# Autodesk Inventor assembly: right drive
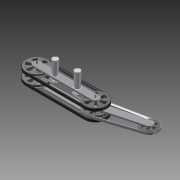
[picture p0: Inventor's stored thumbnail of the model, 180x180]
Saved by Autodesk Inventor 2011 (Build 150239000, 239)
## iProperties
Created: 2010-04-20
Part Number: right drive
Document SubType Name: Assembly
Designer: lucio
Author: lucio
## Documents named in this file (9)
- C:\Users\lucio\Documents\Inventor\caterpillar\right drive.iam
- C:\Users\lucio\Documents\Inventor\caterpillar\base side.ipt
- C:\Users\lucio\Documents\Inventor\caterpillar\mr85vel 2 etapas.ipt
- C:\Users\lucio\Documents\Inventor\caterpillar\mr85vel 3 etapas.ipt
- C:\Users\lucio\Documents\Inventor\caterpillar\back wheel.iam
- C:\Users\lucio\Documents\Inventor\caterpillar\sprocket.ipt
- C:\Users\lucio\Documents\Inventor\caterpillar\chain.ipt
- C:\Users\lucio\Documents\Inventor\caterpillar\big belt.ipt
- C:\Users\lucio\Documents\Inventor\caterpillar\outer drive side.ipt
## Components (11 placed, 8 different names)
1. base side:1 — Insert:1, Insert:2, Insert:4
2. mr85vel 2 etapas:1 — Insert:1, Mate:2, Flush:2
3. mr85vel 3 etapas:1 — Insert:2, Flush:1, Mate:1
4. back wheel:1 [sub-assembly] — Insert:4, Mate:7, Mate:10, Mate:11, Mate:14
5. sprocket:1 — Flush:1, Mate:1, Mate:4, Mate:3
6. sprocket:2 — Mate:2, Flush:2, Mate:8, Mate:6
7. chain:1 — Mate:4, Mate:3
8. chain:2 — Mate:8, Mate:7, Mate:6
9. big belt:1 — Mate:10
10. big belt:2 — Mate:11
11. outer drive side:1 — Mate:14
## Relationships (15: Mate 8, Flush 4, Insert 3)
- Insert:1: base side:1 ↔ mr85vel 2 etapas:1
- Insert:2: base side:1 ↔ mr85vel 3 etapas:1
- Insert:4 (2 mm): base side:1 ↔ back wheel:1
- Flush:1: mr85vel 3 etapas:1 ↔ sprocket:1
- Mate:1: mr85vel 3 etapas:1 ↔ sprocket:1
- Mate:2: mr85vel 2 etapas:1 ↔ sprocket:2
- Flush:2: mr85vel 2 etapas:1 ↔ sprocket:2
- Mate:4: sprocket:1 ↔ chain:1
- Mate:3 [Flush] (-0.5 mm): sprocket:1 ↔ chain:1
- Mate:8 [Flush]: sprocket:2 ↔ chain:2
- Mate:7: back wheel:1 ↔ chain:2
- Mate:6: sprocket:2 ↔ chain:2
- Mate:10: back wheel:1 ↔ big belt:1
- Mate:11: back wheel:1 ↔ big belt:2
- Mate:14: back wheel:1 ↔ outer drive side:1
